# Autodesk Inventor assembly: 362-50
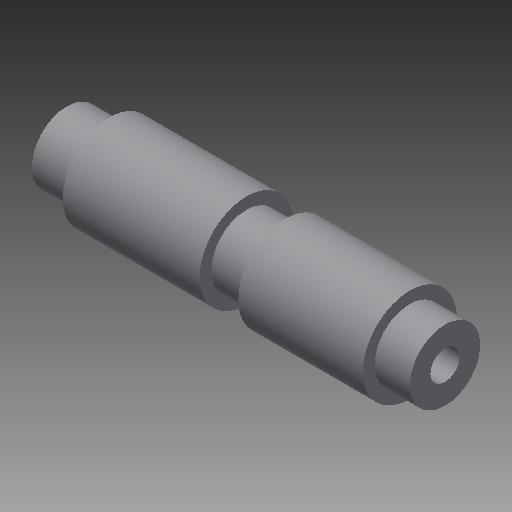
[picture p0: Inventor's stored thumbnail of the model, 512x512]
Saved by Autodesk Inventor 2019 (Build 230136000, 136)
## iProperties
Company: Autodesk Inc.
Created: 2017-03-19
Part Number: 362-50
Document SubType Name: Assembly
Designer: Autodesk Inc.
Mass: 9.944 g
Surface Area: 79.0166 cm^2
Volume: 9.944 cm^3
Density: 1 g/cm^3
Author: Inventor
## Documents named in this file (4)
- C:\TEMP\Jet Engine Model\Workspace\Turbine Link Assembly.iam
- C:\TEMP\Jet Engine Model\Workspace\Turbine Link.ipt
- C:\TEMP\Jet Engine Model\Workspace\Turbine Spacer-6.ipt
- C:\TEMP\Jet Engine Model\Workspace\Turbine Spacer-4.ipt
## Components (3 placed, 3 different names)
1. Turbine Link:1
2. Turbine Spacer-6:1
3. Turbine Spacer-4:1
## Relationships (3: Mate 3)
- [Mate]: Turbine Link:1 ↔ Turbine Spacer-6:1
- [Mate]: Turbine Link:1 ↔ Turbine Spacer-4:1
- [Mate] (6.6 mm): Turbine Spacer-6:1 ↔ Turbine Spacer-4:1
